# Autodesk Inventor assembly: PSI Gauge 1764
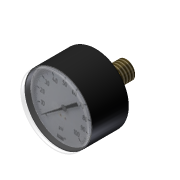
[picture p0: Inventor's stored thumbnail of the model, 180x180]
Saved by Autodesk Inventor 2011 (Build 150239000, 239)
## iProperties
Created: 2010-02-12
Part Number: PSI Gauge 1764
Document SubType Name: Assembly
Designer: jgehrig
Author: jgehrig
## Documents named in this file (5)
- R:\2010-2011\CMO\Web Site\CADalog\Pneumatics\PSI Gage 1764\PSI Gauge 1764.iam
- R:\2010-2011\CMO\Web Site\CADalog\Pneumatics\PSI Gage 1764\PSI Gauge Base 1764.ipt
- R:\2010-2011\CMO\Web Site\CADalog\Pneumatics\PSI Gage 1764\PSI Gauge Screw 1764.ipt
- R:\2010-2011\CMO\Web Site\CADalog\Pneumatics\PSI Gage 1764\PSI Gauge Cap 1764.ipt
- R:\2010-2011\CMO\Web Site\CADalog\Pneumatics\PSI Gage 1764\PSI Guage Face 1764.ipt
## Components (4 placed, 4 different names)
1. PSI Gauge Base 1764:1 — Mate:1, Mate:2, Insert:1, Mate:3, Mate:4
2. PSI Gauge Screw 1764:1 — Mate:3, Mate:4
3. PSI Gauge Cap 1764:1 — Insert:1
4. PSI Guage Face 1764:1 — Mate:1, Mate:2
## Relationships (5: Mate 4, Insert 1)
- Mate:1: PSI Gauge Base 1764:1 ↔ PSI Guage Face 1764:1
- Mate:2 (16.51 mm): PSI Gauge Base 1764:1 ↔ PSI Guage Face 1764:1
- Insert:1: PSI Gauge Base 1764:1 ↔ PSI Gauge Cap 1764:1
- Mate:3: PSI Gauge Base 1764:1 ↔ PSI Gauge Screw 1764:1
- Mate:4: PSI Gauge Base 1764:1 ↔ PSI Gauge Screw 1764:1
